(part 1 of 2)
# Autodesk Inventor assembly: printer
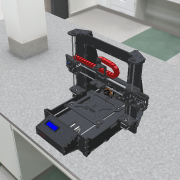
[picture p0: Inventor's stored thumbnail of the model, 180x180]
Saved by Autodesk Inventor 2014 (Build 180170000, 170)
## iProperties
Created: 2014-01-09
Part Number: printer
Document SubType Name: Assembly
Designer: buben
Author: buben
## Documents named in this file (48)
- C:\Users\buben\Documents\GitHub\bacon\inventor files\assemblies\printer.iam
- C:\Users\buben\Documents\GitHub\bacon\inventor files\printer parts\brace_left.ipt
- C:\Users\buben\Documents\GitHub\bacon\inventor files\printer parts\bottom.ipt
- C:\Users\buben\Documents\GitHub\bacon\inventor files\printer parts\brace_right.ipt
- C:\Users\buben\Documents\GitHub\bacon\inventor files\printer parts\front.ipt
- C:\Users\buben\Documents\GitHub\bacon\inventor files\printer parts\back.ipt
- C:\Users\buben\Documents\GitHub\bacon\inventor files\printer parts\frame.ipt
- C:\Users\buben\Documents\GitHub\bacon\inventor files\printer parts\z_motor_brace.ipt
- C:\Users\buben\Documents\GitHub\bacon\inventor files\printer parts\z_motor_mount.ipt
- C:\Users\buben\Documents\GitHub\bacon\inventor files\printer parts\y_axis_cap.ipt
- C:\Users\buben\Documents\GitHub\bacon\inventor files\printer parts\z_rod_stopper_bottom.ipt
- C:\Users\buben\Documents\GitHub\bacon\inventor files\3rd party components\nema_17_stepper\Imported Components\NEMA 17\NEMA 17.iam
- C:\Users\buben\Documents\GitHub\bacon\inventor files\utils\z_axis_rod.ipt
- C:\Users\buben\Documents\GitHub\bacon\inventor files\utils\z_threaded_rod.ipt
- C:\Users\buben\Documents\GitHub\bacon\inventor files\utils\y_axis_rod.ipt
- C:\Users\buben\Documents\GitHub\bacon\inventor files\printer parts\z_axis_top.ipt
- C:\Users\buben\Documents\GitHub\bacon\inventor files\printer parts\z_axis_top_cap.ipt
- C:\Users\buben\Documents\GitHub\bacon\inventor files\printer parts\frame_brace_top.ipt
- C:\Users\buben\Documents\GitHub\bacon\inventor files\utils\washer_m4.ipt
- C:\Users\buben\Documents\Inventor\Content Center Files\R2014\en-US\ISO 4762(2)\ISO 4762 - M4 x 20ISO.ipt
- C:\Users\buben\Documents\Inventor\Content Center Files\R2014\en-US\DIN 985\DIN 985 - M4.ipt
- C:\Users\buben\Documents\Inventor\Content Center Files\R2014\en-US\ISO 7040\ISO 7040 - M4.ipt
- C:\Users\buben\Documents\GitHub\bacon\inventor files\printer parts\wiring_brace.ipt
- C:\Users\buben\Documents\GitHub\bacon\inventor files\utils\washer_m3.ipt
- C:\Users\buben\Documents\Inventor\Content Center Files\R2014\en-US\ISO 4762(2)\ISO 4762 - M3 x 16ISO.ipt
- C:\Users\buben\Documents\GitHub\bacon\inventor files\3rd party components\PC Fan\Imported Components\PC Fan\PC Fan.iam
- C:\Users\buben\Documents\GitHub\bacon\inventor files\3rd party components\fan guard\Imported Components\User Library-Fan Guard\User Library-Fan Guard.ipt
- C:\Users\buben\Documents\GitHub\bacon\inventor files\printer parts\y_carriage_belt_iddler.ipt
- C:\Users\buben\Documents\GitHub\bacon\inventor files\printer parts\y_carriage_belt_iddler_holder.ipt
- C:\Users\buben\Documents\GitHub\bacon\inventor files\3rd party components\bearing_608\Imported Components\608RS\608RS.ipt
- C:\Users\buben\Documents\GitHub\bacon\inventor files\utils\belt_guide.ipt
- C:\Users\buben\Documents\GitHub\bacon\inventor files\utils\washer_m8.ipt
- C:\Users\buben\Documents\Inventor\Content Center Files\R2014\en-US\ISO 7040\ISO 7040 - M8.ipt
- C:\Users\buben\Documents\Inventor\Content Center Files\R2014\en-US\ISO 4762(2)\ISO 4762 - M8 x 40ISO.ipt
- C:\Users\buben\Documents\Inventor\Content Center Files\R2014\en-US\ISO 4762(2)\ISO 4762 - M4 x 30ISO.ipt
- C:\Users\buben\Documents\GitHub\bacon\inventor files\printer parts\y_motor_mount.ipt
- C:\Users\buben\Documents\GitHub\bacon\inventor files\printer parts\y_motor_mount_brace.ipt
- C:\Users\buben\Documents\GitHub\bacon\inventor files\printer parts\motor_spacer.ipt
- C:\Users\buben\Documents\GitHub\bacon\inventor files\3rd party components\nema_17_stepper\Imported Components\NEMA 17 with T5 Pulley\NEMA 17 with T5 Pulley.iam
- C:\Users\buben\Documents\GitHub\bacon\inventor files\assemblies\y_carryage.iam
- C:\Users\buben\Documents\GitHub\bacon\inventor files\assemblies\x_axis.iam
- C:\Users\buben\Documents\Inventor\lcd.ipt
- C:\Users\buben\Documents\GitHub\bacon\inventor files\printer parts\front_panel_2004_display.ipt
- C:\Users\buben\Documents\GitHub\bacon\inventor files\printer parts\front_panel_2004_brace_left.ipt
- C:\Users\buben\Documents\GitHub\bacon\inventor files\printer parts\front_panel_2004_front.ipt
- C:\Users\buben\Documents\GitHub\bacon\inventor files\printer parts\front_panel_2004_bottom.ipt
- C:\Users\buben\Documents\GitHub\bacon\inventor files\printer parts\front_panel_2004_brace_right.ipt
- C:\Users\buben\Documents\GitHub\bacon\inventor files\3rd party components\USB socket\Imported Components\USB-Socket\USB-Socket.ipt
## Components (477 placed, 47 different names)
1. brace_left:1 — Mate:1, Mate:2, Mate:3, Mate:4, Mate:5, Flush:1, Mate:8, Mate:9, Mate:10, Mate:11, Mate:13, Mate:14, Mate:15, Mate:16, Mate:23, Mate:24, Mate:25, Mate:78, Mate:79, Flush:3, Mate:123, Mate:205, Mate:207
2. bottom:1 — Mate:4, Mate:5, Flush:1, Mate:6, Flush:2, Mate:7, Mate:12, Mate:80, Mate:91, Mate:484, Mate:485
3. brace_right:1 — Mate:6, Flush:2, Mate:7, Mate:26, Mate:28, Mate:70, Mate:90, Mate:184, Mate:202, Mate:204, Mate:211, Mate:212, Mate:341, Mate:342, Mate:360
4. front:1 — Mate:8, Mate:9, Mate:10, Mate:29, Mate:30, Mate:31, Mate:32, Mate:33, Mate:34, Mate:84, Mate:85, Mate:86, Mate:87, Mate:134, Mate:135, Mate:304, Mate:305, Mate:306, Mate:307, Mate:308, Mate:309, Mate:310, Mate:402, Mate:403, Flush:7, Mate:415, Mate:430, Mate:431, Mate:432, Mate:433
5. back:1 — Mate:11, Mate:12, Mate:13, Mate:35, Mate:36, Mate:37, Mate:38, Mate:39, Mate:40, Insert:3, Insert:4, Mate:255, Mate:256, Mate:257, Mate:258, Mate:286, Mate:287, Mate:288, Mate:289, Mate:290, Mate:291, Mate:292
6. frame:1 — Mate:14, Mate:15, Mate:16, Mate:17, Mate:18, Mate:19, Mate:20, Mate:21, Mate:22, Mate:27, Mate:57, Mate:58, Mate:59, Mate:60, Mate:61, Mate:62, Mate:69, Mate:71, Flush:4, Mate:121, Mate:122, Mate:168, Mate:169, Mate:170, Mate:171, Mate:172, Mate:173, Mate:203, Mate:206, Mate:208, Mate:209, Mate:362, Mate:364
7. z_motor_brace:1 — Mate:20, Mate:21, Mate:22
8. z_motor_brace:2 — Mate:17, Mate:18, Mate:19, Mate:174, Mate:176
9. z_motor_mount:1 — Mate:23, Mate:24, Mate:25, Mate:44, Mate:45, Mate:46, Mate:52, Insert:2
10. z_motor_mount:2 — Mate:26, Mate:27, Mate:28, Mate:41, Mate:42, Mate:43, Insert:1, Mate:160, Mate:161, Mate:162, Mate:163, Mate:164, Mate:165, Mate:166, Mate:167, Mate:180, Mate:182, Mate:220, Mate:221, Mate:222, Mate:223, Mate:224, Mate:225, Mate:226, Mate:227
11. y_axis_cap:1 — Mate:30, Mate:33, Mate:34
12. y_axis_cap:2 — Mate:35, Mate:39, Mate:40
13. y_axis_cap:3 — Mate:36, Mate:37, Mate:38
14. y_axis_cap:4 — Mate:29, Mate:31, Mate:32, Mate:130, Mate:131, Mate:132, Mate:133
15. z_rod_stopper_bottom:1 — Mate:44, Mate:45, Mate:46, Mate:50, Mate:51
16. z_rod_stopper_bottom:2 — Mate:41, Mate:42, Mate:43, Mate:47, Mate:48, Mate:49, Mate:178, Mate:186
17. NEMA 17:1 [sub-assembly] — Mate:47, Mate:48, Mate:49, Mate:53, Mate:54
18. NEMA 17:2 [sub-assembly] — Mate:50, Mate:51, Mate:52, Mate:55, Mate:56
19. z_axis_rod:1 — Insert:1, Mate:340
20. z_axis_rod:2 — Insert:2, Mate:339
21. z_threaded_rod:1 — Mate:55, Mate:56
22. z_threaded_rod:2 — Mate:53, Mate:54
23. y_axis_rod:1 — Insert:3, Mate:338
24. y_axis_rod:2 — Insert:4, Mate:337
25. z_axis_top:1 — Mate:57, Mate:58, Mate:59, Mate:63, Mate:67, Mate:68
26. z_axis_top:2 — Mate:60, Mate:61, Mate:62, Mate:64, Mate:65, Mate:66, Mate:354, Mate:355, Mate:356, Mate:357, Mate:358, Mate:359, Mate:366, Mate:368
27. z_axis_top_cap:1 — Mate:63, Mate:67, Mate:68
28. z_axis_top_cap:2 — Mate:64, Mate:65, Mate:66, Mate:350, Mate:351, Mate:352, Mate:353
29. frame_brace_top:1 — Mate:69, Mate:70, Mate:71, Mate:343
30. DIN 985 - replaced by DIN EN ISO 10511 M4:12
31. CSN 02 1702 B B 4,3:30 — Insert:9
32. CSN 02 1702 B B 4,3:31 — Mate:106, Mate:108
33. ISO 4762 M4 x 20:15 — Mate:106, Insert:9, Mate:107
34. DIN EN ISO 7040 M4:6 — Mate:107, Mate:108
35. DIN EN ISO 7040 M4:7
36. CSN 02 1702 B B 4,3:32
37. ISO 4762 M4 x 20:16
38. CSN 02 1702 B B 4,3:33
39. DIN EN ISO 7040 M4:8
40. CSN 02 1702 B B 4,3:34
41. ISO 4762 M4 x 20:17
42. CSN 02 1702 B B 4,3:35
43. CSN 02 1702 B B 4,3:42 — Insert:10
44. CSN 02 1702 B B 4,3:43 — Insert:11
45. CSN 02 1702 B B 4,3:44 — Mate:109, Mate:112
46. CSN 02 1702 B B 4,3:45 — Mate:110, Mate:114
47. ISO 4762 M4 x 20:21 — Mate:109, Insert:10, Mate:111
48. ISO 4762 M4 x 20:22 — Mate:110, Insert:11, Mate:113
49. DIN EN ISO 7040 M4:12 — Mate:111, Mate:112
50. DIN EN ISO 7040 M4:13 — Mate:113, Mate:114
51. DIN EN ISO 7040 M4:14
52. CSN 02 1702 B B 4,3:46
53. ISO 4762 M4 x 20:23
54. CSN 02 1702 B B 4,3:47
55. DIN EN ISO 7040 M4:15
56. CSN 02 1702 B B 4,3:48
57. ISO 4762 M4 x 20:24
58. CSN 02 1702 B B 4,3:49
59. CSN 02 1702 B B 4,3:50 — Mate:115, Mate:116
60. ISO 4762 M4 x 20:25 — Mate:115, Mate:117
61. DIN EN ISO 7040 M4:16 — Mate:116, Mate:117
62. DIN EN ISO 7040 M4:17
63. CSN 02 1702 B B 4,3:51
64. ISO 4762 M4 x 20:26
65. CSN 02 1702 B B 4,3:52
66. DIN EN ISO 7040 M4:18
67. CSN 02 1702 B B 4,3:53
68. ISO 4762 M4 x 20:27
69. CSN 02 1702 B B 4,3:54
70. ISO 4762 M4 x 20:28
71. CSN 02 1702 B B 4,3:55
72. CSN 02 1702 B B 4,3:56
73. DIN EN ISO 7040 M4:19
74. ISO 4762 M4 x 20:29
75. CSN 02 1702 B B 4,3:57
76. CSN 02 1702 B B 4,3:58
77. DIN EN ISO 7040 M4:20
78. ISO 4762 M4 x 20:30
79. CSN 02 1702 B B 4,3:59
80. CSN 02 1702 B B 4,3:60
81. DIN EN ISO 7040 M4:21
82. ISO 4762 M4 x 20:35 — Mate:118, Insert:12, Mate:119
83. CSN 02 1702 B B 4,3:69 — Mate:118, Mate:120
84. CSN 02 1702 B B 4,3:70 — Insert:12
85. DIN EN ISO 7040 M4:26 — Mate:119, Mate:120
86. ISO 4762 M4 x 20:36
87. CSN 02 1702 B B 4,3:71
88. CSN 02 1702 B B 4,3:72
89. DIN EN ISO 7040 M4:27
90. ISO 4762 M4 x 20:37
91. CSN 02 1702 B B 4,3:73
92. CSN 02 1702 B B 4,3:74
93. DIN EN ISO 7040 M4:28
94. ISO 4762 M4 x 20:38
95. CSN 02 1702 B B 4,3:75
96. CSN 02 1702 B B 4,3:76
97. DIN EN ISO 7040 M4:29
98. ISO 4762 M4 x 20:39
99. CSN 02 1702 B B 4,3:77
100. CSN 02 1702 B B 4,3:78
101. DIN EN ISO 7040 M4:30
102. CSN 02 1702 B B 4,3:89 — Insert:14
103. CSN 02 1702 B B 4,3:90 — Mate:127, Mate:129
104. ISO 4762 M4 x 20:45 — Mate:127, Insert:14, Mate:128
105. DIN EN ISO 7040 M4:36 — Mate:128, Mate:129
106. ISO 4762 M4 x 20:46
107. CSN 02 1702 B B 4,3:91
108. CSN 02 1702 B B 4,3:92
109. DIN EN ISO 7040 M4:37
110. ISO 4762 M4 x 20:47
111. CSN 02 1702 B B 4,3:93
112. CSN 02 1702 B B 4,3:94
113. DIN EN ISO 7040 M4:38
114. ISO 4762 M4 x 20:48
115. CSN 02 1702 B B 4,3:95
116. CSN 02 1702 B B 4,3:96
117. DIN EN ISO 7040 M4:39
118. ISO 4762 M4 x 20:49
119. CSN 02 1702 B B 4,3:97
120. CSN 02 1702 B B 4,3:98
121. DIN EN ISO 7040 M4:40
122. CSN 02 1702 B B 4,3:99 — Mate:131, Mate:133, Insert:16
123. CSN 02 1702 B B 4,3:100 — Mate:130, Mate:132, Insert:15
124. CSN 02 1702 B B 4,3:101 — Mate:134, Mate:136, Mate:140
125. CSN 02 1702 B B 4,3:102 — Mate:135, Mate:137, Mate:138
126. ISO 4762 M4 x 20:50 — Insert:16, Mate:136, Mate:141
127. ISO 4762 M4 x 20:51 — Insert:15, Mate:137, Mate:139
128. DIN EN ISO 7040 M4:41 — Mate:138, Mate:139
129. DIN EN ISO 7040 M4:42 — Mate:140, Mate:141
130. CSN 02 1702 B B 4,3:103 — Insert:17
131. CSN 02 1702 B B 4,3:104 — Insert:18
132. CSN 02 1702 B B 4,3:105 — Mate:142, Mate:147
133. CSN 02 1702 B B 4,3:106 — Mate:143, Mate:145
134. ISO 4762 M4 x 20:52 — Mate:142, Insert:17, Mate:146
135. ISO 4762 M4 x 20:53 — Mate:143, Insert:18, Mate:144
136. DIN EN ISO 7040 M4:43 — Mate:144, Mate:145
137. DIN EN ISO 7040 M4:44 — Mate:146, Mate:147
138. CSN 02 1702 B B 4,3:107 — Insert:19
139. CSN 02 1702 B B 4,3:108 — Insert:20
140. CSN 02 1702 B B 4,3:109 — Mate:148, Mate:153
141. CSN 02 1702 B B 4,3:110 — Mate:149, Mate:151
142. ISO 4762 M4 x 20:54 — Mate:148, Insert:19, Mate:152
143. ISO 4762 M4 x 20:55 — Mate:149, Insert:20, Mate:150
144. DIN EN ISO 7040 M4:45 — Mate:150, Mate:151
145. DIN EN ISO 7040 M4:46 — Mate:152, Mate:153
146. CSN 02 1702 B B 4,3:111 — Insert:21
147. CSN 02 1702 B B 4,3:112 — Insert:22
148. CSN 02 1702 B B 4,3:113 — Mate:154, Mate:158
149. CSN 02 1702 B B 4,3:114 — Mate:155, Mate:156
150. ISO 4762 M4 x 20:56 — Insert:21, Mate:154, Mate:159
151. ISO 4762 M4 x 20:57 — Insert:22, Mate:155, Mate:157
152. DIN EN ISO 7040 M4:47 — Mate:156, Mate:157
153. DIN EN ISO 7040 M4:48 — Mate:158, Mate:159
154. CSN 02 1702 B B 4,3:115 — Mate:176, Mate:177, Mate:190
155. CSN 02 1702 B B 4,3:116 — Mate:164, Mate:165, Insert:25
156. CSN 02 1702 B B 4,3:117 — Mate:172, Mate:173, Insert:29
157. CSN 02 1702 B B 4,3:118 — Mate:182, Mate:183, Mate:196
158. CSN 02 1702 B B 4,3:119 — Mate:178, Mate:179, Mate:188
159. CSN 02 1702 B B 4,3:120 — Mate:162, Mate:163, Insert:23
160. CSN 02 1702 B B 4,3:121 — Mate:160, Mate:161, Insert:24
161. CSN 02 1702 B B 4,3:122 — Mate:166, Mate:167, Insert:26
162. CSN 02 1702 B B 4,3:123 — Mate:168, Mate:169, Insert:27
163. CSN 02 1702 B B 4,3:124 — Mate:170, Mate:171, Insert:28
164. CSN 02 1702 B B 4,3:125 — Mate:174, Mate:175, Mate:192
165. CSN 02 1702 B B 4,3:126 — Mate:184, Mate:185, Mate:198
166. CSN 02 1702 B B 4,3:127 — Mate:186, Mate:187, Mate:200
167. CSN 02 1702 B B 4,3:128 — Mate:180, Mate:181, Mate:194
168. ISO 4762 M4 x 20:58 — Insert:28, Mate:183, Mate:197
169. ISO 4762 M4 x 20:59 — Insert:29, Mate:175, Mate:193
170. ISO 4762 M4 x 20:60 — Insert:27, Mate:181, Mate:195
171. ISO 4762 M4 x 20:61 — Insert:26, Mate:187, Mate:201
172. ISO 4762 M4 x 20:62 — Insert:25, Mate:185, Mate:199
173. ISO 4762 M4 x 20:63 — Insert:24, Mate:179, Mate:189
174. ISO 4762 M4 x 20:64 — Insert:23, Mate:177, Mate:191
175. DIN EN ISO 7040 M4:49 — Mate:200, Mate:201
176. DIN EN ISO 7040 M4:50 — Mate:198, Mate:199
177. DIN EN ISO 7040 M4:51 — Mate:188, Mate:189
178. DIN EN ISO 7040 M4:52 — Mate:192, Mate:193
179. DIN EN ISO 7040 M4:53 — Mate:194, Mate:195
180. DIN EN ISO 7040 M4:54 — Mate:190, Mate:191
181. DIN EN ISO 7040 M4:55 — Mate:196, Mate:197
182. wiring_brace:1 — Mate:202, Mate:203, Mate:204, Mate:210, Mate:213
183. wiring_brace:2 — Mate:205, Mate:206, Mate:207
184. CSN 02 1702 B B 4,3:129 — Mate:211, Mate:212, Insert:31
185. CSN 02 1702 B B 4,3:130 — Mate:213, Mate:215, Mate:218
186. CSN 02 1702 B B 4,3:131 — Mate:210, Mate:214, Mate:216
187. CSN 02 1702 B B 4,3:132 — Mate:208, Mate:209, Insert:30
188. ISO 4762 M4 x 20:65 — Insert:30, Mate:214, Mate:217
189. ISO 4762 M4 x 20:66 — Insert:31, Mate:215, Mate:219
190. DIN EN ISO 7040 M4:56 — Mate:218, Mate:219
191. DIN EN ISO 7040 M4:57 — Mate:216, Mate:217
192. CSN 02 1702 B B 3,2:1 — Mate:222, Mate:227, Insert:35
193. CSN 02 1702 B B 3,2:2 — Mate:221, Mate:224, Insert:33
194. CSN 02 1702 B B 3,2:3 — Mate:220, Mate:226, Insert:34
195. CSN 02 1702 B B 3,2:4 — Mate:223, Mate:225, Insert:32
196. ISO 4762 M3 x 16:1 — Insert:33
197. ISO 4762 M3 x 16:2 — Insert:32
198. ISO 4762 M3 x 16:3 — Insert:34
199. ISO 4762 M3 x 16:4 — Insert:35
200. CSN 02 1702 B B 4,3:133 — Mate:234, Mate:246
201. CSN 02 1702 B B 4,3:134 — Insert:40
202. CSN 02 1702 B B 4,3:135 — Insert:37
203. CSN 02 1702 B B 4,3:136 — Mate:228, Mate:248
204. CSN 02 1702 B B 4,3:137 — Mate:233, Mate:240
205. CSN 02 1702 B B 4,3:138 — Insert:42
206. CSN 02 1702 B B 4,3:139 — Insert:41
207. CSN 02 1702 B B 4,3:140 — Insert:39
208. CSN 02 1702 B B 4,3:141 — Insert:38
209. CSN 02 1702 B B 4,3:142 — Insert:36
210. CSN 02 1702 B B 4,3:143 — Mate:229, Mate:242
211. CSN 02 1702 B B 4,3:144 — Mate:232, Mate:238
212. CSN 02 1702 B B 4,3:145 — Mate:231, Mate:236
213. CSN 02 1702 B B 4,3:146 — Mate:230, Mate:244
214. ISO 4762 M4 x 20:67 — Mate:228, Insert:36, Mate:247
215. ISO 4762 M4 x 20:68 — Mate:229, Insert:37, Mate:241
216. ISO 4762 M4 x 20:69 — Mate:230, Insert:38, Mate:243
217. ISO 4762 M4 x 20:70 — Mate:231, Insert:39, Mate:235
218. ISO 4762 M4 x 20:71 — Mate:232, Insert:40, Mate:237
219. ISO 4762 M4 x 20:72 — Mate:233, Insert:41, Mate:239
220. ISO 4762 M4 x 20:73 — Mate:234, Insert:42, Mate:245
221. DIN EN ISO 7040 M4:58 — Mate:235, Mate:236
222. DIN EN ISO 7040 M4:59 — Mate:237, Mate:238
223. DIN EN ISO 7040 M4:60 — Mate:239, Mate:240
224. DIN EN ISO 7040 M4:61 — Mate:241, Mate:242
225. DIN EN ISO 7040 M4:62 — Mate:243, Mate:244
226. DIN EN ISO 7040 M4:63 — Mate:245, Mate:246
227. DIN EN ISO 7040 M4:64 — Mate:247, Mate:248
228. CSN 02 1702 B B 4,3:147 — Insert:44
229. CSN 02 1702 B B 4,3:148 — Mate:250, Mate:252
230. CSN 02 1702 B B 4,3:149 — Mate:249, Mate:254
231. CSN 02 1702 B B 4,3:150 — Insert:43
232. ISO 4762 M4 x 20:74 — Mate:249, Insert:43, Mate:253
233. ISO 4762 M4 x 20:75 — Mate:250, Insert:44, Mate:251
234. DIN EN ISO 7040 M4:65 — Mate:251, Mate:252
235. DIN EN ISO 7040 M4:66 — Mate:253, Mate:254
236. CSN 02 1702 B B 3,2:5 — Insert:48
237. CSN 02 1702 B B 3,2:6 — Insert:45
238. CSN 02 1702 B B 3,2:7 — Insert:47
239. CSN 02 1702 B B 3,2:8 — Insert:46
240. ISO 4762 M3 x 16:5 — Insert:45
241. ISO 4762 M3 x 16:6 — Insert:46
242. ISO 4762 M3 x 16:7 — Insert:47
243. ISO 4762 M3 x 16:8 — Insert:48
244. PC Fan:1 [sub-assembly] — Mate:255, Mate:256, Mate:257
245. User Library-Fan Guard:1 — Mate:258
246. y_carriage_belt_iddler:1 — Mate:262, Mate:263, Mate:264, Mate:278, Mate:282, Mate:283, Mate:288
247. y_carriage_belt_iddler:2 — Mate:259, Mate:260, Mate:261, Mate:279, Mate:280, Mate:281, Mate:286, Mate:287
248. y_carriage_belt_iddler_holder:1 — Mate:259, Mate:260, Mate:261, Mate:262, Mate:263, Mate:264, Mate:293, Mate:294
249. 608RS:1 — Mate:265, Mate:266, Mate:269, Mate:274, Mate:275, Mate:276, Mate:277, Mate:279
250. belt_guide:1 — Mate:265, Mate:266, Mate:267, Mate:268
251. belt_guide:2 — Mate:267, Mate:268, Mate:269
252. CSN 02 1702 B B 8,4:1 — Mate:280, Mate:281, Mate:284
253. CSN 02 1702 B B 8,4:2 — Mate:282, Mate:283, Insert:49
254. CSN 02 1702 B B 8,4:3 — Mate:272, Mate:273
255. CSN 02 1702 B B 8,4:4 — Mate:272, Mate:273, Mate:274, Mate:275
256. CSN 02 1702 B B 8,4:5 — Mate:270, Mate:271, Mate:276, Mate:277
257. CSN 02 1702 B B 8,4:6 — Mate:270, Mate:271, Mate:278
258. ISO 4762 M8 x 40:1 — Insert:49, Mate:285
259. DIN EN ISO 7040 M8:1 — Mate:284, Mate:285
260. CSN 02 1702 B B 4,3:151 — Mate:294, Mate:295, Mate:297
261. CSN 02 1702 B B 4,3:152 — Mate:289, Mate:292, Insert:50
262. CSN 02 1702 B B 4,3:153 — Mate:290, Mate:291, Insert:51
263. CSN 02 1702 B B 4,3:154 — Mate:293, Mate:296, Mate:299
264. ISO 4762 M4 x 30:1 — Insert:50, Mate:296, Mate:300
265. ISO 4762 M4 x 30:2 — Insert:51, Mate:295, Mate:298
266. DIN EN ISO 7040 M4:67 — Mate:299, Mate:300
267. DIN EN ISO 7040 M4:68 — Mate:297, Mate:298
268. y_motor_mount:1 — Mate:301, Mate:302, Mate:303, Mate:304, Mate:306, Mate:311, Mate:312, Mate:317, Mate:328, Tangent:1, Tangent:2, Mate:329, Mate:330, Mate:331, Mate:332, Mate:486
269. y_motor_mount_brace:1 — Mate:301, Mate:302, Mate:303, Mate:305, Mate:313, Mate:315
270. CSN 02 1702 B B 4,3:155 — Mate:315, Mate:316, Mate:323
271. CSN 02 1702 B B 4,3:156 — Mate:317, Mate:318, Mate:319
272. CSN 02 1702 B B 4,3:157 — Mate:311, Mate:312, Insert:54
273. CSN 02 1702 B B 4,3:158 — Mate:313, Mate:314, Mate:321
274. CSN 02 1702 B B 4,3:159 — Mate:307, Mate:310, Insert:53
275. CSN 02 1702 B B 4,3:160 — Mate:308, Mate:309, Insert:52
276. ISO 4762 M4 x 20:76 — Insert:54, Mate:316, Mate:324
277. ISO 4762 M4 x 20:77 — Insert:53, Mate:318, Mate:320
278. ISO 4762 M4 x 20:78 — Insert:52, Mate:314, Mate:322
279. DIN EN ISO 7040 M4:69 — Mate:321, Mate:322
280. DIN EN ISO 7040 M4:70 — Mate:319, Mate:320
281. DIN EN ISO 7040 M4:71 — Mate:323, Mate:324
282. motor_spacer:1 — Mate:325, Mate:326, Mate:327, Mate:328, Tangent:1, Tangent:2, Mate:333, Mate:334, Mate:335, Mate:336
283. NEMA 17 with T5 Pulley:1 [sub-assembly] — Mate:325, Mate:326, Mate:327
284. CSN 02 1702 B B 3,2:9 — Mate:331, Insert:57
285. CSN 02 1702 B B 3,2:10 — Mate:332, Insert:58
286. CSN 02 1702 B B 3,2:11 — Mate:330, Insert:56
287. CSN 02 1702 B B 3,2:12 — Mate:329, Insert:55
288. ISO 4762 M3 x 16:9 — Insert:58, Mate:335
289. ISO 4762 M3 x 16:10 — Insert:57, Mate:336
290. ISO 4762 M3 x 16:11 — Insert:56, Mate:334
291. ISO 4762 M3 x 16:12 — Insert:55, Mate:333
292. y_carryage:1 [sub-assembly] — Mate:337, Mate:338
293. x_axis:1 [sub-assembly] — Mate:339, Mate:340
294. CSN 02 1702 B B 4,3:161 — Mate:341, Mate:342, Insert:59
295. CSN 02 1702 B B 4,3:162 — Mate:343, Mate:344, Mate:345
296. ISO 4762 M4 x 20:79 — Insert:59, Mate:344, Mate:346
297. DIN EN ISO 7040 M4:72 — Mate:345, Mate:346
298. CSN 02 1702 B B 4,3:163 — Insert:60
299. CSN 02 1702 B B 4,3:164 — Mate:347, Mate:349
300. ISO 4762 M4 x 20:80 — Mate:347, Insert:60, Mate:348
301. DIN EN ISO 7040 M4:73 — Mate:348, Mate:349
302. CSN 02 1702 B B 4,3:165 — Mate:362, Mate:363, Mate:373
303. CSN 02 1702 B B 4,3:166 — Mate:364, Mate:365, Mate:371
304. CSN 02 1702 B B 4,3:167 — Mate:366, Mate:367, Mate:375
305. CSN 02 1702 B B 4,3:168 — Mate:368, Mate:377, Mate:378
306. CSN 02 1702 B B 4,3:169 — Mate:360, Mate:361, Mate:369
307. CSN 02 1702 B B 4,3:170 — Mate:356, Mate:357, Insert:61
308. CSN 02 1702 B B 4,3:171 — Mate:355, Mate:359, Insert:62
309. CSN 02 1702 B B 4,3:172 — Mate:350, Mate:353, Insert:65
310. CSN 02 1702 B B 4,3:173 — Mate:354, Mate:358, Insert:63
311. CSN 02 1702 B B 4,3:174 — Mate:351, Mate:352, Insert:64
312. ISO 4762 M4 x 20:81 — Insert:61, Mate:361, Mate:370
313. ISO 4762 M4 x 20:82 — Insert:62, Mate:365, Mate:372
314. ISO 4762 M4 x 20:83 — Insert:63, Mate:363, Mate:374
315. ISO 4762 M4 x 20:84 — Insert:64, Mate:367, Mate:376
316. ISO 4762 M4 x 20:85 — Insert:65, Mate:378, Mate:379
317. DIN EN ISO 7040 M4:74 — Mate:377, Mate:379
318. DIN EN ISO 7040 M4:75 — Mate:375, Mate:376
319. DIN EN ISO 7040 M4:76 — Mate:373, Mate:374
320. DIN EN ISO 7040 M4:77 — Mate:371, Mate:372
321. DIN EN ISO 7040 M4:78 — Mate:369, Mate:370
322. CSN 02 1702 B B 4,3:175 — Mate:382, Mate:390
323. CSN 02 1702 B B 4,3:176 — Mate:381, Mate:392
324. CSN 02 1702 B B 4,3:177 — Mate:383, Mate:388
325. CSN 02 1702 B B 4,3:178 — Mate:384, Mate:386
326. CSN 02 1702 B B 4,3:179 — Mate:380, Mate:394
327. CSN 02 1702 B B 4,3:180 — Insert:66
328. CSN 02 1702 B B 4,3:181 — Insert:67
329. CSN 02 1702 B B 4,3:182 — Insert:70
330. CSN 02 1702 B B 4,3:183 — Insert:68
331. CSN 02 1702 B B 4,3:184 — Insert:69
332. ISO 4762 M4 x 20:86 — Mate:380, Insert:66, Mate:393
333. ISO 4762 M4 x 20:87 — Mate:381, Insert:67, Mate:391
334. ISO 4762 M4 x 20:88 — Mate:382, Insert:68, Mate:389
335. ISO 4762 M4 x 20:89 — Mate:383, Insert:69, Mate:387
336. ISO 4762 M4 x 20:90 — Mate:384, Insert:70, Mate:385
337. DIN EN ISO 7040 M4:79 — Mate:385, Mate:386
338. DIN EN ISO 7040 M4:80 — Mate:387, Mate:388
339. DIN EN ISO 7040 M4:81 — Mate:389, Mate:390
340. DIN EN ISO 7040 M4:82 — Mate:391, Mate:392
341. DIN EN ISO 7040 M4:83 — Mate:393, Mate:394
342. lcd:1 — Flush:8, Mate:404, Mate:405
343. front_panel_2004_brace_left:1 — Mate:402, Mate:403, Flush:7, Mate:406, Mate:407, Mate:408, Mate:409, Mate:410, Mate:411, Mate:412, Mate:413, Mate:414
344. front_panel_2004_display:1 — Flush:8, Mate:404, Mate:405, Mate:406, Mate:407, Mate:408, Mate:416, Mate:417, Mate:434, Mate:436, Mate:438
345. front_panel_2004_front:1 — Mate:409, Mate:410, Mate:411, Mate:440, Mate:490, Mate:491, Mate:492, Mate:493, Mate:494, Mate:495
346. front_panel_2004_bottom:1 — Mate:412, Mate:413, Mate:414, Mate:446, Mate:448
347. front_panel_2004_brace_right:1 — Mate:415, Mate:416, Mate:417, Mate:418, Mate:419, Mate:420, Mate:421, Mate:422, Mate:423, Mate:424, Mate:425, Mate:426, Mate:427, Mate:428, Mate:429, Mate:442, Mate:444
348. CSN 02 1702 B B 4,3:185 — Mate:440, Mate:441, Mate:454
349. CSN 02 1702 B B 4,3:186 — Mate:432, Mate:433, Insert:77
350. CSN 02 1702 B B 4,3:187 — Mate:436, Mate:437, Mate:458
351. CSN 02 1702 B B 4,3:188 — Mate:438, Mate:439, Mate:456
352. CSN 02 1702 B B 4,3:189 — Mate:444, Mate:445, Mate:464
353. CSN 02 1702 B B 4,3:190 — Mate:448, Mate:449, Mate:450
354. CSN 02 1702 B B 4,3:191 — Mate:446, Mate:447, Mate:452
355. CSN 02 1702 B B 4,3:192 — Mate:442, Mate:443, Mate:462
356. CSN 02 1702 B B 4,3:193 — Mate:434, Mate:435, Mate:460
357. CSN 02 1702 B B 4,3:194 — Mate:430, Mate:431, Insert:78
358. CSN 02 1702 B B 4,3:195 — Mate:428, Mate:429, Insert:74
359. CSN 02 1702 B B 4,3:196 — Mate:426, Mate:427, Insert:73
360. CSN 02 1702 B B 4,3:197 — Mate:424, Mate:425, Insert:71
361. CSN 02 1702 B B 4,3:198 — Mate:422, Mate:423, Insert:76
362. CSN 02 1702 B B 4,3:199 — Mate:418, Mate:419, Insert:72
363. CSN 02 1702 B B 4,3:200 — Mate:420, Mate:421, Insert:75
364. ISO 4762 M4 x 20:91 — Insert:71, Mate:441, Mate:455
365. ISO 4762 M4 x 20:92 — Insert:74, Mate:449, Mate:451
366. ISO 4762 M4 x 20:93 — Insert:75, Mate:437, Mate:459
367. ISO 4762 M4 x 20:94 — Insert:76, Mate:435, Mate:461
368. ISO 4762 M4 x 20:95 — Insert:77, Mate:445, Mate:465
369. ISO 4762 M4 x 20:96 — Insert:78, Mate:443, Mate:463
370. ISO 4762 M4 x 20:97 — Insert:73, Mate:447, Mate:453
371. ISO 4762 M4 x 20:98 — Insert:72, Mate:439, Mate:457
372. DIN EN ISO 7040 M4:84 — Mate:454, Mate:455
373. DIN EN ISO 7040 M4:85 — Mate:452, Mate:453
374. DIN EN ISO 7040 M4:86 — Mate:460, Mate:461
375. DIN EN ISO 7040 M4:87 — Mate:462, Mate:463
376. DIN EN ISO 7040 M4:88 — Mate:464, Mate:465
377. DIN EN ISO 7040 M4:89 — Mate:458, Mate:459
378. DIN EN ISO 7040 M4:90 — Mate:456, Mate:457
379. DIN EN ISO 7040 M4:91 — Mate:450, Mate:451
380. CSN 02 1702 B B 4,3:201 — Mate:466, Mate:473
381. CSN 02 1702 B B 4,3:202 — Insert:81
382. CSN 02 1702 B B 4,3:203 — Mate:471, Mate:481
383. CSN 02 1702 B B 4,3:204 — Mate:468, Mate:479
384. CSN 02 1702 B B 4,3:205 — Mate:467, Mate:483
385. CSN 02 1702 B B 4,3:206 — Mate:470, Mate:475
386. CSN 02 1702 B B 4,3:207 — Mate:469, Mate:477
387. CSN 02 1702 B B 4,3:208 — Insert:82
388. CSN 02 1702 B B 4,3:209 — Insert:80
389. CSN 02 1702 B B 4,3:210 — Insert:83
390. CSN 02 1702 B B 4,3:211 — Insert:79
391. CSN 02 1702 B B 4,3:212 — Insert:84
392. ISO 4762 M4 x 20:99 — Mate:466, Insert:79, Mate:472
393. ISO 4762 M4 x 20:100 — Mate:467, Insert:80, Mate:482
394. ISO 4762 M4 x 20:101 — Mate:468, Insert:81, Mate:478
395. ISO 4762 M4 x 20:102 — Mate:469, Insert:82, Mate:476
396. ISO 4762 M4 x 20:103 — Mate:470, Insert:83, Mate:474
397. ISO 4762 M4 x 20:104 — Mate:471, Insert:84, Mate:480
398. DIN EN ISO 7040 M4:92 — Mate:472, Mate:473
399. DIN EN ISO 7040 M4:93 — Mate:474, Mate:475
400. DIN EN ISO 7040 M4:94 — Mate:476, Mate:477
401. DIN EN ISO 7040 M4:95 — Mate:478, Mate:479
402. DIN EN ISO 7040 M4:96 — Mate:480, Mate:481
403. DIN EN ISO 7040 M4:97 — Mate:482, Mate:483
404. CSN 02 1702 B B 4,3:213 — Mate:484, Mate:485, Insert:85
405. CSN 02 1702 B B 4,3:214 — Mate:486, Mate:487, Mate:488
406. ISO 4762 M4 x 20:105 — Insert:85, Mate:487, Mate:489
407. DIN EN ISO 7040 M4:98 — Mate:488, Mate:489
408. USB-Socket:1 — Mate:490, Mate:492, Mate:495
409. USB-Socket:2 — Mate:491, Mate:493, Mate:494
410. DIN EN ISO 7040 M4:2 — Mate:102, Mate:103
411. CSN 02 1702 B B 4,3:23 — Mate:90, Mate:94, Mate:102
412. ISO 4762 M4 x 20:11 — Insert:7, Mate:94, Mate:103
413. CSN 02 1702 B B 4,3:21 — Mate:84, Mate:85, Insert:7
414. DIN EN ISO 7040 M4:4
415. CSN 02 1702 B B 4,3:26
416. ISO 4762 M4 x 20:13
417. CSN 02 1702 B B 4,3:27
418. DIN EN ISO 7040 M4:5
419. CSN 02 1702 B B 4,3:28
420. ISO 4762 M4 x 20:14
421. CSN 02 1702 B B 4,3:29
422. ISO 4762 M4 x 20:12 — Insert:8, Mate:95, Mate:105
423. CSN 02 1702 B B 4,3:22 — Mate:86, Mate:87, Insert:8
424. CSN 02 1702 B B 4,3:25 — Mate:91, Mate:95, Mate:104
425. DIN EN ISO 7040 M4:3 — Mate:104, Mate:105
426. ISO 4762 M4 x 20:18
427. CSN 02 1702 B B 4,3:36
428. CSN 02 1702 B B 4,3:37
429. DIN EN ISO 7040 M4:9
430. ISO 4762 M4 x 20:19
431. CSN 02 1702 B B 4,3:38
432. CSN 02 1702 B B 4,3:39
433. DIN EN ISO 7040 M4:10
434. ISO 4762 M4 x 20:20
435. CSN 02 1702 B B 4,3:40
436. CSN 02 1702 B B 4,3:41
437. DIN EN ISO 7040 M4:11
438. ISO 4762 M4 x 20:6 — Insert:6, Mate:81, Mate:101
439. CSN 02 1702 B B 4,3:12 — Mate:78, Mate:79, Insert:6
440. CSN 02 1702 B B 4,3:11 — Mate:80, Mate:81, Mate:100
441. DIN EN ISO 7040 M4:1 — Mate:100, Mate:101
442. ISO 4762 M4 x 20:31
443. CSN 02 1702 B B 4,3:61
444. CSN 02 1702 B B 4,3:62
445. DIN EN ISO 7040 M4:22
446. ISO 4762 M4 x 20:32
447. CSN 02 1702 B B 4,3:63
448. CSN 02 1702 B B 4,3:64
449. DIN EN ISO 7040 M4:23
450. ISO 4762 M4 x 20:33
451. CSN 02 1702 B B 4,3:65
452. CSN 02 1702 B B 4,3:66
453. DIN EN ISO 7040 M4:24
454. ISO 4762 M4 x 20:34
455. CSN 02 1702 B B 4,3:67
456. CSN 02 1702 B B 4,3:68
457. DIN EN ISO 7040 M4:25
458. ISO 4762 M4 x 20:40 — Insert:13, Mate:124, Mate:126
459. CSN 02 1702 B B 4,3:79 — Mate:121, Mate:122, Insert:13
460. CSN 02 1702 B B 4,3:80 — Mate:123, Mate:124, Mate:125
461. DIN EN ISO 7040 M4:31 — Mate:125, Mate:126
462. ISO 4762 M4 x 20:41
463. CSN 02 1702 B B 4,3:81
464. CSN 02 1702 B B 4,3:82
465. DIN EN ISO 7040 M4:32
466. ISO 4762 M4 x 20:42
467. CSN 02 1702 B B 4,3:83
468. CSN 02 1702 B B 4,3:84
469. DIN EN ISO 7040 M4:33
470. ISO 4762 M4 x 20:43
471. CSN 02 1702 B B 4,3:85
472. CSN 02 1702 B B 4,3:86
473. DIN EN ISO 7040 M4:34
474. ISO 4762 M4 x 20:44
475. CSN 02 1702 B B 4,3:87
476. CSN 02 1702 B B 4,3:88
477. DIN EN ISO 7040 M4:35
## Component patterns: (3 elements, first: DIN EN ISO 7040 M4:2 + CSN 02 1702 B B 4,3:23 + ISO 4762 M4 x 20:11 + CSN 02 1702 B B 4,3:21), (4 elements, first: ISO 4762 M4 x 20:12 + CSN 02 1702 B B 4,3:22 + CSN 02 1702 B B 4,3:25 + DIN EN ISO 7040 M4:3), (5 elements, first: ISO 4762 M4 x 20:6 + CSN 02 1702 B B 4,3:12 + CSN 02 1702 B B 4,3:11 + DIN EN ISO 7040 M4:1), (5 elements, first: ISO 4762 M4 x 20:40 + CSN 02 1702 B B 4,3:79 + CSN 02 1702 B B 4,3:80 + DIN EN ISO 7040 M4:31)
## Relationships (564: Mate 472, Insert 84, Flush 6, Tangent 2)
- Mate:1: brace_left:1
- Mate:2: brace_left:1
- Mate:3: brace_left:1
- Mate:4: brace_left:1 ↔ bottom:1
- Mate:5: brace_left:1 ↔ bottom:1
- Flush:1: brace_left:1 ↔ bottom:1
- Mate:6: bottom:1 ↔ brace_right:1
- Flush:2: bottom:1 ↔ brace_right:1
- Mate:7: bottom:1 ↔ brace_right:1
- Mate:8: brace_left:1 ↔ front:1
- Mate:9: brace_left:1 ↔ front:1
- Mate:10: brace_left:1 ↔ front:1
- Mate:11: brace_left:1 ↔ back:1
- Mate:12: bottom:1 ↔ back:1
- Mate:13: brace_left:1 ↔ back:1
- Mate:14: brace_left:1 ↔ frame:1
- Mate:15: brace_left:1 ↔ frame:1
- Mate:16: brace_left:1 ↔ frame:1
- Mate:17: frame:1 ↔ z_motor_brace:2
- Mate:18: frame:1 ↔ z_motor_brace:2
- Mate:19: frame:1 ↔ z_motor_brace:2
- Mate:20: frame:1 ↔ z_motor_brace:1
- Mate:21: frame:1 ↔ z_motor_brace:1
- Mate:22: frame:1 ↔ z_motor_brace:1
- Mate:23: brace_left:1 ↔ z_motor_mount:1
- Mate:24: brace_left:1 ↔ z_motor_mount:1
- Mate:25: brace_left:1 ↔ z_motor_mount:1
- Mate:26: brace_right:1 ↔ z_motor_mount:2
- Mate:27: frame:1 ↔ z_motor_mount:2
- Mate:28: brace_right:1 ↔ z_motor_mount:2
- Mate:29: front:1 ↔ y_axis_cap:4
- Mate:30: front:1 ↔ y_axis_cap:1
- Mate:31: front:1 ↔ y_axis_cap:4
- Mate:32: front:1 ↔ y_axis_cap:4
- Mate:33: front:1 ↔ y_axis_cap:1
- Mate:34: front:1 ↔ y_axis_cap:1
- Mate:35: back:1 ↔ y_axis_cap:2
- Mate:36: back:1 ↔ y_axis_cap:3
- Mate:37: back:1 ↔ y_axis_cap:3
- Mate:38: back:1 ↔ y_axis_cap:3
- Mate:39: back:1 ↔ y_axis_cap:2
- Mate:40: back:1 ↔ y_axis_cap:2
- Mate:41: z_motor_mount:2 ↔ z_rod_stopper_bottom:2
- Mate:42: z_motor_mount:2 ↔ z_rod_stopper_bottom:2
- Mate:43: z_motor_mount:2 ↔ z_rod_stopper_bottom:2
- Mate:44: z_motor_mount:1 ↔ z_rod_stopper_bottom:1
- Mate:45: z_motor_mount:1 ↔ z_rod_stopper_bottom:1
- Mate:46: z_motor_mount:1 ↔ z_rod_stopper_bottom:1
- Mate:47: z_rod_stopper_bottom:2 ↔ NEMA 17:1
- Mate:48: z_rod_stopper_bottom:2 ↔ NEMA 17:1
- Mate:49: z_rod_stopper_bottom:2 ↔ NEMA 17:1
- Mate:50: z_rod_stopper_bottom:1 ↔ NEMA 17:2
- Mate:51: z_rod_stopper_bottom:1 ↔ NEMA 17:2
- Mate:52: z_motor_mount:1 ↔ NEMA 17:2
- Insert:1: z_motor_mount:2 ↔ z_axis_rod:1
- Insert:2: z_motor_mount:1 ↔ z_axis_rod:2
- Mate:53: NEMA 17:1 ↔ z_threaded_rod:2
- Mate:54: NEMA 17:1 ↔ z_threaded_rod:2
- Mate:55: NEMA 17:2 ↔ z_threaded_rod:1
- Mate:56: NEMA 17:2 ↔ z_threaded_rod:1
- Insert:3: back:1 ↔ y_axis_rod:1
- Insert:4: back:1 ↔ y_axis_rod:2
- Mate:57: frame:1 ↔ z_axis_top:1
- Mate:58: frame:1 ↔ z_axis_top:1
- Mate:59: frame:1 ↔ z_axis_top:1
- Mate:60: frame:1 ↔ z_axis_top:2
- Mate:61: frame:1 ↔ z_axis_top:2
- Mate:62: frame:1 ↔ z_axis_top:2
- Mate:63: z_axis_top:1 ↔ z_axis_top_cap:1
- Mate:64: z_axis_top:2 ↔ z_axis_top_cap:2
- Mate:65: z_axis_top:2 ↔ z_axis_top_cap:2
- Mate:66: z_axis_top:2 ↔ z_axis_top_cap:2
- Mate:67: z_axis_top:1 ↔ z_axis_top_cap:1
- Mate:68: z_axis_top:1 ↔ z_axis_top_cap:1
- Mate:69: frame:1 ↔ frame_brace_top:1
- Mate:70: brace_right:1 ↔ frame_brace_top:1
- Mate:71: frame:1 ↔ frame_brace_top:1
- Mate:78: brace_left:1 ↔ CSN 02 1702 B B 4,3:12
- Mate:79: brace_left:1 ↔ CSN 02 1702 B B 4,3:12
- Mate:80: bottom:1 ↔ CSN 02 1702 B B 4,3:11
- Insert:6: ISO 4762 M4 x 20:6 ↔ CSN 02 1702 B B 4,3:12
- Mate:81: ISO 4762 M4 x 20:6 ↔ CSN 02 1702 B B 4,3:11
- Mate:84: front:1 ↔ CSN 02 1702 B B 4,3:21
- Mate:85: front:1 ↔ CSN 02 1702 B B 4,3:21
- Mate:86: front:1 ↔ CSN 02 1702 B B 4,3:22
- Mate:87: front:1 ↔ CSN 02 1702 B B 4,3:22
- Mate:90: brace_right:1 ↔ CSN 02 1702 B B 4,3:23
- Mate:91: bottom:1 ↔ CSN 02 1702 B B 4,3:25
- Insert:7: ISO 4762 M4 x 20:11 ↔ CSN 02 1702 B B 4,3:21
- Insert:8: ISO 4762 M4 x 20:12 ↔ CSN 02 1702 B B 4,3:22
- Mate:94: CSN 02 1702 B B 4,3:23 ↔ ISO 4762 M4 x 20:11
- Mate:95: ISO 4762 M4 x 20:12 ↔ CSN 02 1702 B B 4,3:25
- Flush:3 (167.5 mm): brace_left:1
- Mate:100: CSN 02 1702 B B 4,3:11 ↔ DIN EN ISO 7040 M4:1
- Mate:101: ISO 4762 M4 x 20:6 ↔ DIN EN ISO 7040 M4:1
- Mate:102: DIN EN ISO 7040 M4:2 ↔ CSN 02 1702 B B 4,3:23
- Mate:103: DIN EN ISO 7040 M4:2 ↔ ISO 4762 M4 x 20:11
- Mate:104: CSN 02 1702 B B 4,3:25 ↔ DIN EN ISO 7040 M4:3
- Mate:105: ISO 4762 M4 x 20:12 ↔ DIN EN ISO 7040 M4:3
- Flush:4 (77 mm): frame:1
- Mate:106: CSN 02 1702 B B 4,3:31 ↔ ISO 4762 M4 x 20:15
- Insert:9: CSN 02 1702 B B 4,3:30 ↔ ISO 4762 M4 x 20:15
- Mate:107: ISO 4762 M4 x 20:15 ↔ DIN EN ISO 7040 M4:6
- Mate:108: CSN 02 1702 B B 4,3:31 ↔ DIN EN ISO 7040 M4:6
- Mate:109: CSN 02 1702 B B 4,3:44 ↔ ISO 4762 M4 x 20:21
- Insert:10: CSN 02 1702 B B 4,3:42 ↔ ISO 4762 M4 x 20:21
- Mate:110: CSN 02 1702 B B 4,3:45 ↔ ISO 4762 M4 x 20:22
- Insert:11: CSN 02 1702 B B 4,3:43 ↔ ISO 4762 M4 x 20:22
- Mate:111: ISO 4762 M4 x 20:21 ↔ DIN EN ISO 7040 M4:12
- Mate:112: CSN 02 1702 B B 4,3:44 ↔ DIN EN ISO 7040 M4:12
- Mate:113: ISO 4762 M4 x 20:22 ↔ DIN EN ISO 7040 M4:13
- Mate:114: CSN 02 1702 B B 4,3:45 ↔ DIN EN ISO 7040 M4:13
- Mate:115: CSN 02 1702 B B 4,3:50 ↔ ISO 4762 M4 x 20:25
- Mate:116: CSN 02 1702 B B 4,3:50 ↔ DIN EN ISO 7040 M4:16
- Mate:117: ISO 4762 M4 x 20:25 ↔ DIN EN ISO 7040 M4:16
- Mate:118: ISO 4762 M4 x 20:35 ↔ CSN 02 1702 B B 4,3:69
- Insert:12: ISO 4762 M4 x 20:35 ↔ CSN 02 1702 B B 4,3:70
- Mate:119: ISO 4762 M4 x 20:35 ↔ DIN EN ISO 7040 M4:26
- Mate:120: CSN 02 1702 B B 4,3:69 ↔ DIN EN ISO 7040 M4:26
- Mate:121: frame:1 ↔ CSN 02 1702 B B 4,3:79
- Mate:122: frame:1 ↔ CSN 02 1702 B B 4,3:79
- Insert:13: ISO 4762 M4 x 20:40 ↔ CSN 02 1702 B B 4,3:79
- Mate:123: brace_left:1 ↔ CSN 02 1702 B B 4,3:80
- Mate:124: ISO 4762 M4 x 20:40 ↔ CSN 02 1702 B B 4,3:80
- Mate:125: CSN 02 1702 B B 4,3:80 ↔ DIN EN ISO 7040 M4:31
- Mate:126: ISO 4762 M4 x 20:40 ↔ DIN EN ISO 7040 M4:31
- Mate:127: CSN 02 1702 B B 4,3:90 ↔ ISO 4762 M4 x 20:45
- Insert:14: CSN 02 1702 B B 4,3:89 ↔ ISO 4762 M4 x 20:45
- Mate:128: ISO 4762 M4 x 20:45 ↔ DIN EN ISO 7040 M4:36
- Mate:129: CSN 02 1702 B B 4,3:90 ↔ DIN EN ISO 7040 M4:36
- Mate:130: y_axis_cap:4 ↔ CSN 02 1702 B B 4,3:100
- Mate:131: y_axis_cap:4 ↔ CSN 02 1702 B B 4,3:99
- Mate:132: y_axis_cap:4 ↔ CSN 02 1702 B B 4,3:100
- Mate:133: y_axis_cap:4 ↔ CSN 02 1702 B B 4,3:99
- Mate:134: front:1 ↔ CSN 02 1702 B B 4,3:101
- Mate:135: front:1 ↔ CSN 02 1702 B B 4,3:102
- Insert:15: CSN 02 1702 B B 4,3:100 ↔ ISO 4762 M4 x 20:51
- Insert:16: CSN 02 1702 B B 4,3:99 ↔ ISO 4762 M4 x 20:50
- Mate:136: CSN 02 1702 B B 4,3:101 ↔ ISO 4762 M4 x 20:50
- Mate:137: CSN 02 1702 B B 4,3:102 ↔ ISO 4762 M4 x 20:51
- Mate:138: CSN 02 1702 B B 4,3:102 ↔ DIN EN ISO 7040 M4:41
- Mate:139: ISO 4762 M4 x 20:51 ↔ DIN EN ISO 7040 M4:41
- Mate:140: CSN 02 1702 B B 4,3:101 ↔ DIN EN ISO 7040 M4:42
- Mate:141: ISO 4762 M4 x 20:50 ↔ DIN EN ISO 7040 M4:42
- Mate:142: CSN 02 1702 B B 4,3:105 ↔ ISO 4762 M4 x 20:52
- Insert:17: CSN 02 1702 B B 4,3:103 ↔ ISO 4762 M4 x 20:52
- Mate:143: CSN 02 1702 B B 4,3:106 ↔ ISO 4762 M4 x 20:53
- Insert:18: CSN 02 1702 B B 4,3:104 ↔ ISO 4762 M4 x 20:53
- Mate:144: ISO 4762 M4 x 20:53 ↔ DIN EN ISO 7040 M4:43
- Mate:145: CSN 02 1702 B B 4,3:106 ↔ DIN EN ISO 7040 M4:43
- Mate:146: ISO 4762 M4 x 20:52 ↔ DIN EN ISO 7040 M4:44
- Mate:147: CSN 02 1702 B B 4,3:105 ↔ DIN EN ISO 7040 M4:44
- Mate:148: CSN 02 1702 B B 4,3:109 ↔ ISO 4762 M4 x 20:54
- Insert:19: CSN 02 1702 B B 4,3:107 ↔ ISO 4762 M4 x 20:54
- Mate:149: CSN 02 1702 B B 4,3:110 ↔ ISO 4762 M4 x 20:55
- Insert:20: CSN 02 1702 B B 4,3:108 ↔ ISO 4762 M4 x 20:55
- Mate:150: ISO 4762 M4 x 20:55 ↔ DIN EN ISO 7040 M4:45
- Mate:151: CSN 02 1702 B B 4,3:110 ↔ DIN EN ISO 7040 M4:45
- Mate:152: ISO 4762 M4 x 20:54 ↔ DIN EN ISO 7040 M4:46
- Mate:153: CSN 02 1702 B B 4,3:109 ↔ DIN EN ISO 7040 M4:46
- Insert:21: CSN 02 1702 B B 4,3:111 ↔ ISO 4762 M4 x 20:56
- Mate:154: CSN 02 1702 B B 4,3:113 ↔ ISO 4762 M4 x 20:56
- Insert:22: CSN 02 1702 B B 4,3:112 ↔ ISO 4762 M4 x 20:57
- Mate:155: CSN 02 1702 B B 4,3:114 ↔ ISO 4762 M4 x 20:57
- Mate:156: CSN 02 1702 B B 4,3:114 ↔ DIN EN ISO 7040 M4:47
- Mate:157: ISO 4762 M4 x 20:57 ↔ DIN EN ISO 7040 M4:47
- Mate:158: CSN 02 1702 B B 4,3:113 ↔ DIN EN ISO 7040 M4:48
- Mate:159: ISO 4762 M4 x 20:56 ↔ DIN EN ISO 7040 M4:48
- Mate:160: z_motor_mount:2 ↔ CSN 02 1702 B B 4,3:121
- Mate:161: z_motor_mount:2 ↔ CSN 02 1702 B B 4,3:121
- Mate:162: z_motor_mount:2 ↔ CSN 02 1702 B B 4,3:120
- Mate:163: z_motor_mount:2 ↔ CSN 02 1702 B B 4,3:120
- Mate:164: z_motor_mount:2 ↔ CSN 02 1702 B B 4,3:116
- Mate:165: z_motor_mount:2 ↔ CSN 02 1702 B B 4,3:116